# Autodesk Inventor assembly: Assembled Water Sensor Chassi
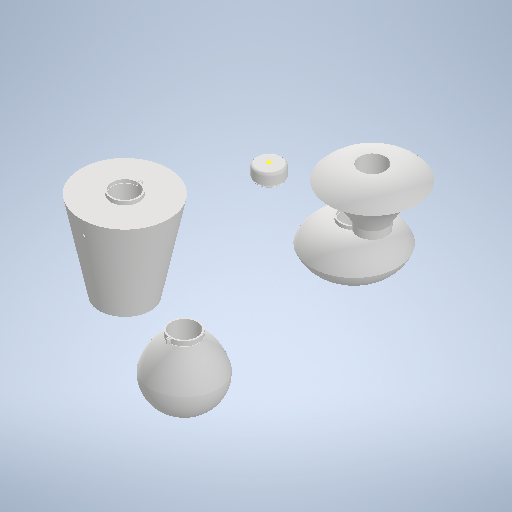
[picture p0: Inventor's stored thumbnail of the model, 512x512]
Saved by Autodesk Inventor 2025 (Build 290162000, 162)
## iProperties
Created: 2024-06-24
Part Number: Assembled Water Sensor Chassi
Document SubType Name: Assembly
Designer: track
Author: track
## Documents named in this file (7)
- C:\Users\track\OneDrive\Documents\In-Situ-Water-Quality-Sensor\System_development\Jocassee\V0.4.7\Bouy_CAD_File\Assembled Water Sensor Chassi.iam
- C:\Users\track\OneDrive\Documents\In-Situ-Water-Quality-Sensor\System_development\Jocassee\V0.4.7\Bouy_CAD_File\Water Sensor Shaft.ipt
- C:\Users\track\OneDrive\Documents\In-Situ-Water-Quality-Sensor\System_development\Jocassee\V0.4.7\Bouy_CAD_File\Water Sensor Bouy 3.ipt
- C:\Users\track\OneDrive\Documents\In-Situ-Water-Quality-Sensor\System_development\Jocassee\V0.4.7\Bouy_CAD_File\Water_Sensor_Cap.ipt
- C:\Users\track\OneDrive\Documents\In-Situ-Water-Quality-Sensor\System_development\Jocassee\V0.4.7\Bouy_CAD_File\Water Sensor Bouy 4.ipt
- C:\Users\track\OneDrive\Documents\In-Situ-Water-Quality-Sensor\System_development\Jocassee\V0.4.7\Bouy_CAD_File\Water Sensor Bouy 1.ipt
- C:\Users\track\OneDrive\Documents\In-Situ-Water-Quality-Sensor\System_development\Jocassee\V0.4.7\Bouy_CAD_File\Water Sensor Bouy 2.ipt
## Components (6 placed, 6 different names)
1. Water Sensor Shaft:1 — Mate:2
2. Water Sensor Bouy 3:1
3. Water_Sensor_Cap:1 — Mate:2
4. Water Sensor Bouy 4:1
5. Water Sensor Bouy 1:1
6. Water Sensor Bouy 2:1
## Relationships (1: Mate 1)
- Mate:2: Water Sensor Shaft:1 ↔ Water_Sensor_Cap:1
